# Autodesk Inventor assembly: Robot
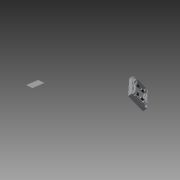
[picture p0: Inventor's stored thumbnail of the model, 180x180]
Saved by Autodesk Inventor 2014 (Build 180170000, 170)
## iProperties
Created: 2014-01-21
Part Number: Robot
Document SubType Name: Assembly
Designer: NilesStanton
Author: NilesStanton
## Documents named in this file (10)
- C:\GitHub\team3566-2014\CAD\Robot.iam
- C:\FIRST-2014-KOP\Drive Base Kit\2014 Sidings.ipt
- C:\FIRST-2014-KOP\Motors\MOT_CIM-Motor_217-2000.iam
- C:\FIRST-2014-KOP\Additions\Flat Board.ipt
- C:\FIRST-2014-KOP\Additions\Front Paneling.ipt
- C:\FIRST-2014-KOP\Additions\3.5 in spacer.ipt
- C:\FIRST-2014-KOP\Additions\Mechanum Wheel.ipt
- C:\FIRST-2014-KOP\Additions\Gearbox.ipt
- C:\FIRST-2014-KOP\Additions\Long Bumber Wood.ipt
- C:\FIRST-2014-KOP\Additions\Short Bumper Wood.ipt
## Components (26 placed, 9 different names)
1. 2014 Sidings:1 — Flush:8, Mate:4, Angle:5, Flush:19, Flush:37, Flush:38
2. 2014 Sidings:2 — Mate:3, Flush:3, Angle:3, Flush:11, Flush:14, Flush:15, Tangent:7, Tangent:8, Flush:22, Flush:23, Flush:25, Flush:26, Flush:30, Flush:31
3. MOT_CIM-Motor_217-2000:1 [sub-assembly] — Tangent:9, Flush:30, Tangent:10
4. MOT_CIM-Motor_217-2000:2 [sub-assembly] — Flush:31, Tangent:11, Tangent:12
5. MOT_CIM-Motor_217-2000:3 [sub-assembly] — Flush:33, Tangent:15, Tangent:16
6. MOT_CIM-Motor_217-2000:4 [sub-assembly] — Flush:32, Tangent:13, Tangent:14
7. Flat Board:1
8. 2014 Sidings:3
9. Front Paneling:1 — Mate:2, Flush:2, Angle:2, Mate:3, Flush:3, Angle:3, Flush:24, Flush:27, Tangent:9, Tangent:15, Mate:7
10. Front Paneling:2 — Mate:1, Flush:1, Angle:1, Flush:5, Flush:7, Flush:9, Flush:10, Flush:18, Flush:21, Tangent:12, Tangent:13, Flush:36, Flush:39, Mate:6
11. 3.5 in spacer:1 — Flush:9, Flush:10, Flush:11, Flush:12, Flush:13, Mate:5, Angle:6, Tangent:1, Tangent:2
12. 3.5 in spacer:2 — Flush:5, Flush:6, Angle:4, Flush:7, Flush:8, Mate:4, Angle:5, Tangent:3, Tangent:4
13. 2014 Sidings:4 — Flush:12, Flush:13, Mate:5, Angle:6, Flush:34, Flush:35
14. 2014 Sidings:5 — Mate:1, Flush:1, Angle:1, Mate:2, Flush:2, Angle:2, Flush:6, Angle:4, Flush:16, Flush:17, Tangent:5, Tangent:6, Flush:20, Flush:28, Flush:29, Flush:32, Flush:33
15. Mechanum Wheel:1 — Flush:14, Tangent:1, Tangent:7
16. Mechanum Wheel:2 — Flush:17, Tangent:4, Tangent:5
17. Mechanum Wheel:3 — Flush:15, Tangent:2, Tangent:8
18. Mechanum Wheel:4 — Flush:16, Tangent:3, Tangent:6
19. Gearbox:1 — Flush:27, Flush:28, Flush:29, Tangent:16
20. Gearbox:2 — Flush:24, Flush:25, Flush:26, Tangent:10
21. Gearbox:3 — Flush:18, Flush:19, Flush:20, Tangent:14
22. Gearbox:4 — Flush:21, Flush:22, Flush:23, Tangent:11
23. Long Bumber Wood:1 — Flush:34, Flush:35, Flush:36, Flush:43, Flush:44
24. Long Bumber Wood:2 — Flush:37, Flush:38, Flush:39, Flush:41, Flush:42
25. Short Bumper Wood:1 — Flush:41, Mate:6, Flush:42
26. Short Bumper Wood:2 — Mate:7, Flush:43, Flush:44
## Relationships (71: Flush 42, Tangent 16, Mate 7, Angle 6)
- Mate:1: Front Paneling:2 ↔ 2014 Sidings:5
- Flush:1: Front Paneling:2 ↔ 2014 Sidings:5
- Angle:1 (90 deg): Front Paneling:2 ↔ 2014 Sidings:5
- Mate:2: Front Paneling:1 ↔ 2014 Sidings:5
- Flush:2: Front Paneling:1 ↔ 2014 Sidings:5
- Angle:2 (90 deg): Front Paneling:1 ↔ 2014 Sidings:5
- Mate:3: 2014 Sidings:2 ↔ Front Paneling:1
- Flush:3: 2014 Sidings:2 ↔ Front Paneling:1
- Angle:3 (90 deg): 2014 Sidings:2 ↔ Front Paneling:1
- Flush:5: Front Paneling:2 ↔ 3.5 in spacer:2
- Flush:6: 3.5 in spacer:2 ↔ 2014 Sidings:5
- Angle:4 (90 deg): 3.5 in spacer:2 ↔ 2014 Sidings:5
- Flush:7: Front Paneling:2 ↔ 3.5 in spacer:2
- Flush:8: 2014 Sidings:1 ↔ 3.5 in spacer:2
- Mate:4: 2014 Sidings:1 ↔ 3.5 in spacer:2
- Angle:5 (90 deg): 2014 Sidings:1 ↔ 3.5 in spacer:2
- Flush:9: Front Paneling:2 ↔ 3.5 in spacer:1
- Flush:10: Front Paneling:2 ↔ 3.5 in spacer:1
- Flush:11: 2014 Sidings:2 ↔ 3.5 in spacer:1
- Flush:12: 3.5 in spacer:1 ↔ 2014 Sidings:4
- Flush:13: 3.5 in spacer:1 ↔ 2014 Sidings:4
- Mate:5: 3.5 in spacer:1 ↔ 2014 Sidings:4
- Angle:6 (90 deg): 3.5 in spacer:1 ↔ 2014 Sidings:4
- Flush:14: 2014 Sidings:2 ↔ Mechanum Wheel:1
- Flush:15: 2014 Sidings:2 ↔ Mechanum Wheel:3
- Tangent:1 (50.8 mm): 3.5 in spacer:1 ↔ Mechanum Wheel:1
- Tangent:2 (622.3 mm): 3.5 in spacer:1 ↔ Mechanum Wheel:3
- Flush:16: 2014 Sidings:5 ↔ Mechanum Wheel:4
- Flush:17: 2014 Sidings:5 ↔ Mechanum Wheel:2
- Tangent:3 (50.8 mm): 3.5 in spacer:2 ↔ Mechanum Wheel:4
- Tangent:4 (622.3 mm): 3.5 in spacer:2 ↔ Mechanum Wheel:2
- Tangent:5 (-38.1 mm): 2014 Sidings:5 ↔ Mechanum Wheel:2
- Tangent:6 (-38.1 mm): 2014 Sidings:5 ↔ Mechanum Wheel:4
- Tangent:7 (-38.1 mm): 2014 Sidings:2 ↔ Mechanum Wheel:1
- Tangent:8 (-38.1 mm): 2014 Sidings:2 ↔ Mechanum Wheel:3
- Flush:18 (88.9 mm): Front Paneling:2 ↔ Gearbox:3
- Flush:19 (18.796 mm): 2014 Sidings:1 ↔ Gearbox:3
- Flush:20 (6.35 mm): 2014 Sidings:5 ↔ Gearbox:3
- Flush:21 (88.9 mm): Front Paneling:2 ↔ Gearbox:4
- Flush:22 (6.35 mm): 2014 Sidings:2 ↔ Gearbox:4
- Flush:23 (19.05 mm): 2014 Sidings:2 ↔ Gearbox:4
- Flush:24 (88.9 mm): Front Paneling:1 ↔ Gearbox:2
- Flush:25 (6.35 mm): 2014 Sidings:2 ↔ Gearbox:2
- Flush:26 (19.05 mm): 2014 Sidings:2 ↔ Gearbox:2
- Flush:27 (88.9 mm): Front Paneling:1 ↔ Gearbox:1
- Flush:28 (19.05 mm): 2014 Sidings:5 ↔ Gearbox:1
- Flush:29 (6.35 mm): 2014 Sidings:5 ↔ Gearbox:1
- Tangent:9 (215.9 mm): MOT_CIM-Motor_217-2000:1 ↔ Front Paneling:1
- Flush:30 (44.45 mm): 2014 Sidings:2 ↔ MOT_CIM-Motor_217-2000:1
- Tangent:10 (6.35 mm): MOT_CIM-Motor_217-2000:1 ↔ Gearbox:2
- Flush:31 (44.45 mm): 2014 Sidings:2 ↔ MOT_CIM-Motor_217-2000:2
- Tangent:11 (6.35 mm): MOT_CIM-Motor_217-2000:2 ↔ Gearbox:4
- Tangent:12 (215.9 mm): MOT_CIM-Motor_217-2000:2 ↔ Front Paneling:2
- Flush:32 (44.45 mm): MOT_CIM-Motor_217-2000:4 ↔ 2014 Sidings:5
- Tangent:13 (215.9 mm): MOT_CIM-Motor_217-2000:4 ↔ Front Paneling:2
- Tangent:14 (6.35 mm): MOT_CIM-Motor_217-2000:4 ↔ Gearbox:3
- Flush:33 (44.45 mm): MOT_CIM-Motor_217-2000:3 ↔ 2014 Sidings:5
- Tangent:15 (215.9 mm): MOT_CIM-Motor_217-2000:3 ↔ Front Paneling:1
- Tangent:16 (6.35 mm): MOT_CIM-Motor_217-2000:3 ↔ Gearbox:1
- Flush:34 (6.35 mm): 2014 Sidings:4 ↔ Long Bumber Wood:1
- Flush:35 (-76.2 mm): 2014 Sidings:4 ↔ Long Bumber Wood:1
- Flush:36: Front Paneling:2 ↔ Long Bumber Wood:1
- Flush:37 (6.35 mm): 2014 Sidings:1 ↔ Long Bumber Wood:2
- Flush:38 (-76.2 mm): 2014 Sidings:1 ↔ Long Bumber Wood:2
- Flush:39: Front Paneling:2 ↔ Long Bumber Wood:2
- Flush:41: Long Bumber Wood:2 ↔ Short Bumper Wood:1
- Mate:6: Front Paneling:2 ↔ Short Bumper Wood:1
- Flush:42: Long Bumber Wood:2 ↔ Short Bumper Wood:1
- Mate:7: Front Paneling:1 ↔ Short Bumper Wood:2
- Flush:43: Long Bumber Wood:1 ↔ Short Bumper Wood:2
- Flush:44: Long Bumber Wood:1 ↔ Short Bumper Wood:2
